# Autodesk Inventor assembly: Macroboard
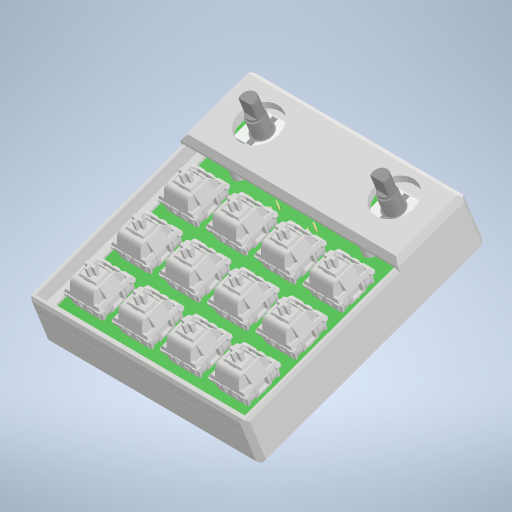
[picture p0: Inventor's stored thumbnail of the model, 512x512]
Saved by Autodesk Inventor 2023.1 (Build 271208000, 208)
## iProperties
Created: 2023-03-16
Part Number: Macroboard
Document SubType Name: Assembly
Designer: nikla
Author: nikla
## Documents named in this file (7)
- C:\Users\nikla\GitHub\MacroBoard\MacroBoard_16keys\3D-model\Macroboard.iam
- C:\Users\nikla\GitHub\MacroBoard\arduino-pro-micro-1.snapshot.1\ARDUINO PRO MICRO.ipt
- C:\Users\nikla\OneDrive\Inventor\3d-Models\cherry-mx-1.snapshot.3\asm_mx_asm_PCB.ipt
- C:\Users\nikla\OneDrive\Inventor\3d-Models\rotary-encoder-17.snapshot.2\旋转编码器.ipt
- C:\Users\nikla\GitHub\MacroBoard\MacroBoard_16keys\3D-model\Bottom.ipt
- C:\Users\nikla\GitHub\MacroBoard\MacroBoard_16keys\3D-model\Top.ipt
- C:\Users\nikla\GitHub\MacroBoard\MacroBoard_16keys\MacroBoard_16keys_v3.ipt
## Components (18 placed, 6 different names)
1. ARDUINO PRO MICRO:1 — Passend:13, Passend:14
2. Bottom:1 — Fluchtend:2, Passend:15
3. Top:1 — Fluchtend:2
4. MacroBoard_16keys_v3:1 — Passend:10, Passend:11, Passend:12, Passend:13, Passend:14, Passend:15
5. asm_mx_asm_PCB:1
6. asm_mx_asm_PCB:2
7. asm_mx_asm_PCB:3
8. asm_mx_asm_PCB:4
9. asm_mx_asm_PCB:5
10. asm_mx_asm_PCB:6
11. asm_mx_asm_PCB:7
12. asm_mx_asm_PCB:8
13. asm_mx_asm_PCB:9
14. asm_mx_asm_PCB:10
15. asm_mx_asm_PCB:11
16. asm_mx_asm_PCB:12
17. 旋转编码器:1 — Passend:10, Passend:11, Passend:12
18. 旋转编码器:2
## Component patterns: (12 elements, first: asm_mx_asm_PCB:1), (2 elements, first: 旋转编码器:1)
## Relationships (10: Mate 9, Flush 1)
- Fluchtend:2 [Flush]: Bottom:1 ↔ Top:1
- [Mate]: ARDUINO PRO MICRO:1 ↔ MacroBoard_16keys_v3:1
- [Mate]: Bottom:1 ↔ MacroBoard_16keys_v3:1
- [Mate]: Bottom:1 ↔ MacroBoard_16keys_v3:1
- Passend:10 [Mate]: MacroBoard_16keys_v3:1 ↔ 旋转编码器:1
- Passend:11 [Mate] (-18.7 mm): MacroBoard_16keys_v3:1 ↔ 旋转编码器:1
- Passend:12 [Mate]: MacroBoard_16keys_v3:1 ↔ 旋转编码器:1
- Passend:13 [Mate]: ARDUINO PRO MICRO:1 ↔ MacroBoard_16keys_v3:1
- Passend:14 [Mate]: ARDUINO PRO MICRO:1 ↔ MacroBoard_16keys_v3:1
- Passend:15 [Mate]: Bottom:1 ↔ MacroBoard_16keys_v3:1
